# Autodesk Inventor assembly: PowerSwitchBoard
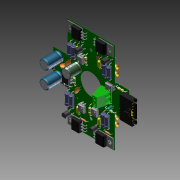
[picture p0: Inventor's stored thumbnail of the model, 180x180]
Saved by Autodesk Inventor 2012 (Build 160160000, 160)
## iProperties
Created: 2014-07-11
Part Number: PowerSwitchBoard
Document SubType Name: Assembly
Designer: Anon
Translation Standard: STEP AP214IS
FileName: Open CASCADE Shape Model
PreProcessor: Open CASCADE 6.2
PostProcessor: Build: 160, Release: 2012 RTM - Date: Tue 03/01/2011
Sent Units: millimeter
Uncertainty: 0.01
Author: Anon
## Documents named in this file (57)
- D:\Dropbox\Courses\GP\Inventor\dronestructure\electronics\powerswitch\PowerSwitchBoard.iam
- D:\Dropbox\Courses\GP\Inventor\dronestructure\electronics\powerswitch\powerswitchpcb\PowerSwitchBoard.ipt
- D:\Dropbox\Courses\GP\Inventor\dronestructure\electronics\powerswitch\powerswitchpcb\T2_SwitchTurbine4.iam
- D:\Dropbox\Courses\GP\Inventor\dronestructure\electronics\powerswitch\powerswitchpcb\T2_SwitchTurbine3.iam
- D:\Dropbox\Courses\GP\Inventor\dronestructure\electronics\powerswitch\powerswitchpcb\T2_SwitchTurbine2.iam
- D:\Dropbox\Courses\GP\Inventor\dronestructure\electronics\powerswitch\powerswitchpcb\T2_SwitchTurbine1.iam
- D:\Dropbox\Courses\GP\Inventor\dronestructure\electronics\powerswitch\powerswitchpcb\T1_SwitchTurbine4.iam
- D:\Dropbox\Courses\GP\Inventor\dronestructure\electronics\powerswitch\powerswitchpcb\T1_SwitchTurbine3.iam
- D:\Dropbox\Courses\GP\Inventor\dronestructure\electronics\powerswitch\powerswitchpcb\T1_SwitchTurbine2.iam
- D:\Dropbox\Courses\GP\Inventor\dronestructure\electronics\powerswitch\powerswitchpcb\T1_SwitchTurbine1.iam
- D:\Dropbox\Courses\GP\Inventor\dronestructure\electronics\powerswitch\powerswitchpcb\R6_SwitchTurbine4.iam
- D:\Dropbox\Courses\GP\Inventor\dronestructure\electronics\powerswitch\powerswitchpcb\R6_SwitchTurbine3.iam
- D:\Dropbox\Courses\GP\Inventor\dronestructure\electronics\powerswitch\powerswitchpcb\R6_SwitchTurbine2.iam
- D:\Dropbox\Courses\GP\Inventor\dronestructure\electronics\powerswitch\powerswitchpcb\R6_SwitchTurbine1.iam
- D:\Dropbox\Courses\GP\Inventor\dronestructure\electronics\powerswitch\powerswitchpcb\R5_SwitchTurbine4.iam
- D:\Dropbox\Courses\GP\Inventor\dronestructure\electronics\powerswitch\powerswitchpcb\R5_SwitchTurbine3.iam
- D:\Dropbox\Courses\GP\Inventor\dronestructure\electronics\powerswitch\powerswitchpcb\R5_SwitchTurbine2.iam
- D:\Dropbox\Courses\GP\Inventor\dronestructure\electronics\powerswitch\powerswitchpcb\R5_SwitchTurbine1.iam
- D:\Dropbox\Courses\GP\Inventor\dronestructure\electronics\powerswitch\powerswitchpcb\R4_SwitchTurbine4.iam
- D:\Dropbox\Courses\GP\Inventor\dronestructure\electronics\powerswitch\powerswitchpcb\R4_SwitchTurbine3.iam
- D:\Dropbox\Courses\GP\Inventor\dronestructure\electronics\powerswitch\powerswitchpcb\R4_SwitchTurbine2.iam
- D:\Dropbox\Courses\GP\Inventor\dronestructure\electronics\powerswitch\powerswitchpcb\R4_SwitchTurbine1.iam
- D:\Dropbox\Courses\GP\Inventor\dronestructure\electronics\powerswitch\powerswitchpcb\IC2_SwitchTurbine4.iam
- D:\Dropbox\Courses\GP\Inventor\dronestructure\electronics\powerswitch\powerswitchpcb\IC2_SwitchTurbine3.iam
- D:\Dropbox\Courses\GP\Inventor\dronestructure\electronics\powerswitch\powerswitchpcb\IC2_SwitchTurbine2.iam
- D:\Dropbox\Courses\GP\Inventor\dronestructure\electronics\powerswitch\powerswitchpcb\IC2_SwitchTurbine1.iam
- D:\Dropbox\Courses\GP\Inventor\dronestructure\electronics\powerswitch\powerswitchpcb\D4_SwitchTurbine4.iam
- D:\Dropbox\Courses\GP\Inventor\dronestructure\electronics\powerswitch\powerswitchpcb\D4_SwitchTurbine3.iam
- D:\Dropbox\Courses\GP\Inventor\dronestructure\electronics\powerswitch\powerswitchpcb\D4_SwitchTurbine2.iam
- D:\Dropbox\Courses\GP\Inventor\dronestructure\electronics\powerswitch\powerswitchpcb\D4_SwitchTurbine1.iam
- D:\Dropbox\Courses\GP\Inventor\dronestructure\electronics\powerswitch\powerswitchpcb\C7_SwitchTurbine4.iam
- D:\Dropbox\Courses\GP\Inventor\dronestructure\electronics\powerswitch\powerswitchpcb\C7_SwitchTurbine3.iam
- D:\Dropbox\Courses\GP\Inventor\dronestructure\electronics\powerswitch\powerswitchpcb\C7_SwitchTurbine2.iam
- D:\Dropbox\Courses\GP\Inventor\dronestructure\electronics\powerswitch\powerswitchpcb\C7_SwitchTurbine1.iam
- D:\Dropbox\Courses\GP\Inventor\dronestructure\electronics\powerswitch\powerswitchpcb\K2.iam
- D:\Dropbox\Courses\GP\Inventor\dronestructure\electronics\powerswitch\powerswitchpcb\K3.iam
- D:\Dropbox\Courses\GP\Inventor\dronestructure\electronics\powerswitch\powerswitchpcb\K4.iam
- D:\Dropbox\Courses\GP\Inventor\dronestructure\electronics\powerswitch\powerswitchpcb\K5.iam
- D:\Dropbox\Courses\GP\Inventor\dronestructure\electronics\powerswitch\powerswitchpcb\K7.iam
- D:\Dropbox\Courses\GP\Inventor\dronestructure\electronics\powerswitch\powerswitchpcb\K8.iam
- D:\Dropbox\Courses\GP\Inventor\dronestructure\electronics\powerswitch\powerswitchpcb\K9.iam
- D:\Dropbox\Courses\GP\Inventor\dronestructure\electronics\powerswitch\powerswitchpcb\K10.iam
- D:\Dropbox\Courses\GP\Inventor\dronestructure\electronics\powerswitch\powerswitchpcb\C1.iam
- D:\Dropbox\Courses\GP\Inventor\dronestructure\electronics\powerswitch\powerswitchpcb\C2.iam
- D:\Dropbox\Courses\GP\Inventor\dronestructure\electronics\powerswitch\powerswitchpcb\C3.iam
- D:\Dropbox\Courses\GP\Inventor\dronestructure\electronics\powerswitch\powerswitchpcb\C4.iam
- D:\Dropbox\Courses\GP\Inventor\dronestructure\electronics\powerswitch\powerswitchpcb\C5.iam
- D:\Dropbox\Courses\GP\Inventor\dronestructure\electronics\powerswitch\powerswitchpcb\C6.iam
- D:\Dropbox\Courses\GP\Inventor\dronestructure\electronics\powerswitch\powerswitchpcb\D1.iam
- D:\Dropbox\Courses\GP\Inventor\dronestructure\electronics\powerswitch\powerswitchpcb\D2.iam
- D:\Dropbox\Courses\GP\Inventor\dronestructure\electronics\powerswitch\powerswitchpcb\D3.iam
- D:\Dropbox\Courses\GP\Inventor\dronestructure\electronics\powerswitch\powerswitchpcb\IC1.iam
- D:\Dropbox\Courses\GP\Inventor\dronestructure\electronics\powerswitch\powerswitchpcb\K1.iam
- D:\Dropbox\Courses\GP\Inventor\dronestructure\electronics\powerswitch\powerswitchpcb\K6.iam
- D:\Dropbox\Courses\GP\Inventor\dronestructure\electronics\powerswitch\powerswitchpcb\R1.iam
- D:\Dropbox\Courses\GP\Inventor\dronestructure\electronics\powerswitch\powerswitchpcb\R2.iam
- D:\Dropbox\Courses\GP\Inventor\dronestructure\electronics\powerswitch\powerswitchpcb\R3.iam
## Components (56 placed, 56 different names)
1. PowerSwitchBoard:1
2. T2_SwitchTurbine4:1 [sub-assembly]
3. T2_SwitchTurbine3:1 [sub-assembly]
4. T2_SwitchTurbine2:1 [sub-assembly]
5. T2_SwitchTurbine1:1 [sub-assembly]
6. T1_SwitchTurbine4:1 [sub-assembly]
7. T1_SwitchTurbine3:1 [sub-assembly]
8. T1_SwitchTurbine2:1 [sub-assembly]
9. T1_SwitchTurbine1:1 [sub-assembly]
10. R6_SwitchTurbine4:1 [sub-assembly]
11. R6_SwitchTurbine3:1 [sub-assembly]
12. R6_SwitchTurbine2:1 [sub-assembly]
13. R6_SwitchTurbine1:1 [sub-assembly]
14. R5_SwitchTurbine4:1 [sub-assembly]
15. R5_SwitchTurbine3:1 [sub-assembly]
16. R5_SwitchTurbine2:1 [sub-assembly]
17. R5_SwitchTurbine1:1 [sub-assembly]
18. R4_SwitchTurbine4:1 [sub-assembly]
19. R4_SwitchTurbine3:1 [sub-assembly]
20. R4_SwitchTurbine2:1 [sub-assembly]
21. R4_SwitchTurbine1:1 [sub-assembly]
22. IC2_SwitchTurbine4:1 [sub-assembly]
23. IC2_SwitchTurbine3:1 [sub-assembly]
24. IC2_SwitchTurbine2:1 [sub-assembly]
25. IC2_SwitchTurbine1:1 [sub-assembly]
26. D4_SwitchTurbine4:1 [sub-assembly]
27. D4_SwitchTurbine3:1 [sub-assembly]
28. D4_SwitchTurbine2:1 [sub-assembly]
29. D4_SwitchTurbine1:1 [sub-assembly]
30. C7_SwitchTurbine4:1 [sub-assembly]
31. C7_SwitchTurbine3:1 [sub-assembly]
32. C7_SwitchTurbine2:1 [sub-assembly]
33. C7_SwitchTurbine1:1 [sub-assembly]
34. K2:1 [sub-assembly]
35. K3:1 [sub-assembly]
36. K4:1 [sub-assembly]
37. K5:1 [sub-assembly]
38. K7:1 [sub-assembly]
39. K8:1 [sub-assembly]
40. K9:1 [sub-assembly]
41. K10:1 [sub-assembly]
42. C1:1 [sub-assembly] — Flush:1
43. C2:1 [sub-assembly]
44. C3:1 [sub-assembly]
45. C4:1 [sub-assembly]
46. C5:1 [sub-assembly]
47. C6:1 [sub-assembly]
48. D1:1 [sub-assembly]
49. D2:1 [sub-assembly]
50. D3:1 [sub-assembly]
51. IC1:1 [sub-assembly]
52. K1:1 [sub-assembly]
53. K6:1 [sub-assembly]
54. R1:1 [sub-assembly]
55. R2:1 [sub-assembly]
56. R3:1 [sub-assembly]
## Relationships (1: Flush 1)
- Flush:1 (-13 mm): C1:1
